# Autodesk Inventor assembly: Conjunto_Inferior
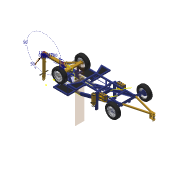
[picture p0: Inventor's stored thumbnail of the model, 180x180]
Saved by Autodesk Inventor 2020 (Build 240168000, 168)
## iProperties
Created: 2020-02-06
Part Number: Conjunto_Inferior
Document SubType Name: Assembly
Designer: Juan Carlos Botero
Author: Juan Carlos Botero
## Documents named in this file (7)
- D:\Drives\OneDrive\Carlos_2\02 TRABAJOS\MULTIPLO\Conveyor\ENSAMBLE\Conjunto_Inferior.iam
- D:\Drives\OneDrive\Carlos_2\02 TRABAJOS\MULTIPLO\Conveyor\ENSAMBLE\Chasis inferior _1_.iam
- D:\Drives\OneDrive\Carlos_2\02 TRABAJOS\MULTIPLO\Conveyor\ENSAMBLE\Eje trasero _1_.iam
- D:\Drives\OneDrive\Carlos_2\02 TRABAJOS\MULTIPLO\Conveyor\ENSAMBLE\Eje delantero _1_.iam
- D:\Drives\OneDrive\Carlos_2\02 TRABAJOS\MULTIPLO\Conveyor\ENSAMBLE\Accesorios.iam
- D:\Drives\OneDrive\Carlos_2\02 TRABAJOS\MULTIPLO\Conveyor\ENSAMBLE\Beacon _1_.iam
- D:\Drives\OneDrive\Carlos_2\02 TRABAJOS\MULTIPLO\Conveyor\ENSAMBLE\Luz _1_.iam
## Components (6 placed, 6 different names)
1. Chasis inferior <1>:1 [sub-assembly] — Mate:1, Mate:2, Mate:3, Rotational:1
2. Eje trasero <1>:1 [sub-assembly]
3. Eje delantero <1>:1 [sub-assembly]
4. Accesorios:1 [sub-assembly]
5. Beacon _1_:1 [sub-assembly] — Mate:1, Mate:2, Mate:3
6. Luz _1_:1 [sub-assembly] — Rotational:1
## Relationships (4: Mate 3, RevoluteJoint 1)
- Mate:1: Chasis inferior <1>:1 ↔ Beacon _1_:1
- Mate:2: Chasis inferior <1>:1 ↔ Beacon _1_:1
- Mate:3: Chasis inferior <1>:1 ↔ Beacon _1_:1
- Rotational:1 [RevoluteJoint] (-2 mm): Chasis inferior <1>:1 ↔ Luz _1_:1
